# Autodesk Inventor assembly: Cartridge
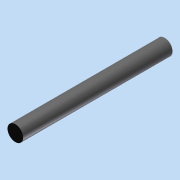
[picture p0: Inventor's stored thumbnail of the model, 180x180]
Saved by Autodesk Inventor 2012 (Build 160160000, 160)
## iProperties
Created: 2015-03-28
Part Number: Cartridge
Document SubType Name: Assembly
Designer: Jason
Author: Jason
## Documents named in this file (3)
- C:\Users\Jason\Documents\Dropbox\Synio\Synio Spray Pen\Product Design\CAD\Markers\Sharpie Fine Point\Cartridge.iam
- C:\Users\Jason\Documents\Dropbox\Synio\Synio Spray Pen\Product Design\CAD\Markers\Sharpie Fine Point\Cartridge-Plastic.ipt
- C:\Users\Jason\Documents\Dropbox\Synio\Synio Spray Pen\Product Design\CAD\Markers\Sharpie Fine Point\Cartridge-Foam.ipt
## Components (2 placed, 2 different names)
1. Cartridge-Plastic:1 — Insert:1
2. Cartridge-Foam:1 — Insert:1
## Relationships (1: Insert 1)
- Insert:1: Cartridge-Plastic:1 ↔ Cartridge-Foam:1
